# Autodesk Inventor assembly: Badminton racket_Final
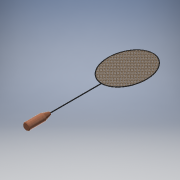
[picture p0: Inventor's stored thumbnail of the model, 180x180]
Saved by Autodesk Inventor 2017 (Build 210142000, 142)
## iProperties
Created: 2016-12-30
Part Number: Badminton racket_Final
Document SubType Name: Assembly
Designer: COEP
Author: COEP
## Documents named in this file (3)
- C:\Users\COEP\Desktop\Badminton racket_Final.iam
- C:\Users\COEP\Desktop\Badminton racket.ipt
- C:\Users\COEP\Desktop\Badminton racket_2.ipt
## Components (2 placed, 2 different names)
1. Badminton racket:1 — Mate:1, Mate:2
2. Badminton racket_2:1 — Mate:1, Mate:2
## Relationships (2: Mate 2)
- Mate:1: Badminton racket:1 ↔ Badminton racket_2:1
- Mate:2: Badminton racket:1 ↔ Badminton racket_2:1
